# Autodesk Inventor assembly: HbHand
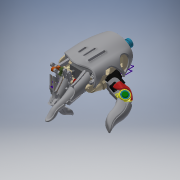
[picture p0: Inventor's stored thumbnail of the model, 180x180]
Saved by Autodesk Inventor 2017 (Build 210142000, 142)
## iProperties
Part Number: HbHand
Material: 一般
Document SubType Name: Assembly
Designer: sktom
Author: sktom
## Documents named in this file (20)
- D:\OneDrive\CAD\hackberry\HACKberry-hardware\3D_69%\HbHand\HbHand.iam
- D:\OneDrive\CAD\hackberry\HACKberry-hardware\3D_69%\HbHand\HbPalmBase03ForChild.ipt
- D:\OneDrive\CAD\hackberry\HACKberry-hardware\3D_69%\HbHand\HbWristMount01ForChild.ipt
- D:\OneDrive\CAD\hackberry\HACKberry-hardware\3D_69%\HbHand\DummyUsmBearing01.ipt
- D:\OneDrive\CAD\hackberry\HACKberry-hardware\3D_69%\HbHand\DummyASV-15MGSingleHorn01.ipt
- D:\OneDrive\CAD\hackberry\HACKberry-hardware\3D_69%\HbHand\HbthumbU02ForChild\HbthumbU02ForChild.iam
- D:\OneDrive\CAD\hackberry\HACKberry-hardware\3D_69%\HbHand\HbFinger01ForChild\HbFinger01ForChild.iam
- D:\OneDrive\CAD\hackberry\HACKberry-hardware\3D_69%\HbHand\HbShaftStopperB04ForChild.ipt
- D:\OneDrive\CAD\hackberry\HACKberry-hardware\3D_69%\HbHand\HbFingerMainCouplerLink01ForChild.ipt
- D:\OneDrive\CAD\hackberry\HACKberry-hardware\3D_69%\HbHand\DummyMetalCollarPh3L5.ipt
- D:\OneDrive\CAD\hackberry\HACKberry-hardware\3D_69%\HbHand\HbMiddle-RingCouplerLink01ForChild.ipt
- D:\OneDrive\CAD\hackberry\HACKberry-hardware\3D_69%\HbHand\HbRing-LittleCouplerLink01ForChild.ipt
- D:\OneDrive\CAD\hackberry\HACKberry-hardware\3D_69%\HbHand\HbIndexFinger01ForChild\HbIndexFinger01ForChild.iam
- D:\OneDrive\CAD\hackberry\HACKberry-hardware\3D_69%\HbHand\HbShaftStopperA04ForChild.ipt
- D:\OneDrive\CAD\hackberry\HACKberry-hardware\3D_69%\HbHand\DummyGWS_S03N.ipt
- D:\OneDrive\CAD\hackberry\HACKberry-hardware\3D_69%\HbHand\DummyHbServoHorn01.ipt
- D:\OneDrive\CAD\hackberry\HACKberry-hardware\3D_69%\HbHand\HbIndexMotorGear02ForChild.ipt
- D:\OneDrive\CAD\hackberry\HACKberry-hardware\3D_69%\HbHand\HbMotorHolder01ForChild.ipt
- D:\OneDrive\CAD\hackberry\HACKberry-hardware\3D_69%\HbHand\DummyASV-15MG.ipt
- D:\OneDrive\CAD\hackberry\HACKberry-hardware\3D_69%\HbHand\HbBackCover02ForChild.ipt
## Components (27 placed, 19 different names)
1. HbPalmBase03ForChild:1 — 挿入:1, 挿入:2, 挿入:3, 挿入:4, 挿入:5, 挿入:7, 円柱状:1, 挿入:8, 円柱状:2, 挿入:9, 円柱状:3, 挿入:10, 挿入:21, 挿入:22, 挿入:26, 挿入:27, 挿入:30, 挿入:31, 挿入:33, 挿入:34
2. HbWristMount01ForChild:1 — 挿入:1, 挿入:2
3. DummyUsmBearing01:1 — 挿入:3
4. DummyASV-15MGSingleHorn01:1 — 挿入:4, 挿入:5, 挿入:6
5. HbthumbU02ForChild:1 [sub-assembly] — 挿入:6
6. HbFinger01ForChild:1 [sub-assembly] — 挿入:7, 円柱状:1, 挿入:13, 円柱状:5
7. HbFinger01ForChild:2 [sub-assembly] — 挿入:8, 円柱状:2, 挿入:18, 挿入:20
8. HbFinger01ForChild:3 [sub-assembly] — 挿入:9, 円柱状:3, 円柱状:4
9. HbShaftStopperB04ForChild:1 — 挿入:10
10. HbFingerMainCouplerLink01ForChild:1 — 挿入:11, 挿入:12
11. DummyMetalCollarPh3L5:1 — 挿入:11, 挿入:13
12. DummyMetalCollarPh3L5:2 — 挿入:12, 円柱状:6
13. DummyMetalCollarPh3L5:3 — 挿入:16, 円柱状:5
14. DummyMetalCollarPh3L5:4 — 挿入:17, 挿入:18
15. DummyMetalCollarPh3L5:5 — 挿入:19, 挿入:20
16. DummyMetalCollarPh3L5:6 — 挿入:15, 円柱状:4
17. HbMiddle-RingCouplerLink01ForChild:1 — 挿入:15, 挿入:19
18. HbRing-LittleCouplerLink01ForChild:1 — 挿入:16, 挿入:17
19. HbIndexFinger01ForChild:1 [sub-assembly] — 挿入:21
20. HbShaftStopperA04ForChild:1 — 挿入:22
21. DummyGWS_S03N:1 — 挿入:25, 挿入:26, 挿入:27
22. DummyHbServoHorn01:1 — 挿入:23, 挿入:24, 挿入:25
23. HbIndexMotorGear02ForChild:1 — 挿入:23, 挿入:24
24. HbMotorHolder01ForChild:1 — 挿入:28, 挿入:29, 挿入:30, 挿入:31
25. DummyASV-15MG:1 — 挿入:28, 挿入:29, 挿入:32
26. DummyASV-15MGSingleHorn01:2 — 挿入:32, 円柱状:6
27. HbBackCover02ForChild:1 — 挿入:33, 挿入:34
## Relationships (39: Insert 33, CylindricalJoint 6)
- 挿入:1 [Insert]: HbPalmBase03ForChild:1 ↔ HbWristMount01ForChild:1
- 挿入:2 [Insert]: HbPalmBase03ForChild:1 ↔ HbWristMount01ForChild:1
- 挿入:3 [Insert]: HbPalmBase03ForChild:1 ↔ DummyUsmBearing01:1
- 挿入:4 [Insert]: HbPalmBase03ForChild:1 ↔ DummyASV-15MGSingleHorn01:1
- 挿入:5 [Insert]: HbPalmBase03ForChild:1 ↔ DummyASV-15MGSingleHorn01:1
- 挿入:6 [Insert]: DummyASV-15MGSingleHorn01:1 ↔ HbthumbU02ForChild:1
- 挿入:7 [Insert] (0.5 mm): HbPalmBase03ForChild:1 ↔ HbFinger01ForChild:1
- 円柱状:1 [CylindricalJoint]: HbPalmBase03ForChild:1 ↔ HbFinger01ForChild:1
- 挿入:8 [Insert] (0.5 mm): HbPalmBase03ForChild:1 ↔ HbFinger01ForChild:2
- 円柱状:2 [CylindricalJoint]: HbPalmBase03ForChild:1 ↔ HbFinger01ForChild:2
- 挿入:9 [Insert] (0.5 mm): HbPalmBase03ForChild:1 ↔ HbFinger01ForChild:3
- 円柱状:3 [CylindricalJoint]: HbPalmBase03ForChild:1 ↔ HbFinger01ForChild:3
- 挿入:10 [Insert]: HbPalmBase03ForChild:1 ↔ HbShaftStopperB04ForChild:1
- 挿入:11 [Insert] (-0.5 mm): HbFingerMainCouplerLink01ForChild:1 ↔ DummyMetalCollarPh3L5:1
- 挿入:12 [Insert] (-0.5 mm): HbFingerMainCouplerLink01ForChild:1 ↔ DummyMetalCollarPh3L5:2
- 挿入:13 [Insert]: HbFinger01ForChild:1 ↔ DummyMetalCollarPh3L5:1
- 挿入:15 [Insert] (-0.2 mm): DummyMetalCollarPh3L5:6 ↔ HbMiddle-RingCouplerLink01ForChild:1
- 挿入:16 [Insert]: DummyMetalCollarPh3L5:3 ↔ HbRing-LittleCouplerLink01ForChild:1
- 挿入:17 [Insert]: DummyMetalCollarPh3L5:4 ↔ HbRing-LittleCouplerLink01ForChild:1
- 挿入:18 [Insert]: HbFinger01ForChild:2 ↔ DummyMetalCollarPh3L5:4
- 挿入:19 [Insert]: DummyMetalCollarPh3L5:5 ↔ HbMiddle-RingCouplerLink01ForChild:1
- 挿入:20 [Insert]: HbFinger01ForChild:2 ↔ DummyMetalCollarPh3L5:5
- 円柱状:4 [CylindricalJoint]: HbFinger01ForChild:3 ↔ DummyMetalCollarPh3L5:6
- 円柱状:5 [CylindricalJoint]: HbFinger01ForChild:1 ↔ DummyMetalCollarPh3L5:3
- 挿入:21 [Insert] (0.25 mm): HbPalmBase03ForChild:1 ↔ HbIndexFinger01ForChild:1
- 挿入:22 [Insert]: HbPalmBase03ForChild:1 ↔ HbShaftStopperA04ForChild:1
- 挿入:23 [Insert]: DummyHbServoHorn01:1 ↔ HbIndexMotorGear02ForChild:1
- 挿入:24 [Insert]: DummyHbServoHorn01:1 ↔ HbIndexMotorGear02ForChild:1
- 挿入:25 [Insert]: DummyGWS_S03N:1 ↔ DummyHbServoHorn01:1
- 挿入:26 [Insert]: HbPalmBase03ForChild:1 ↔ DummyGWS_S03N:1
- 挿入:27 [Insert]: HbPalmBase03ForChild:1 ↔ DummyGWS_S03N:1
- 挿入:28 [Insert]: HbMotorHolder01ForChild:1 ↔ DummyASV-15MG:1
- 挿入:29 [Insert]: HbMotorHolder01ForChild:1 ↔ DummyASV-15MG:1
- 挿入:30 [Insert]: HbPalmBase03ForChild:1 ↔ HbMotorHolder01ForChild:1
- 挿入:31 [Insert]: HbPalmBase03ForChild:1 ↔ HbMotorHolder01ForChild:1
- 挿入:32 [Insert]: DummyASV-15MG:1 ↔ DummyASV-15MGSingleHorn01:2
- 円柱状:6 [CylindricalJoint]: DummyMetalCollarPh3L5:2 ↔ DummyASV-15MGSingleHorn01:2
- 挿入:33 [Insert]: HbPalmBase03ForChild:1 ↔ HbBackCover02ForChild:1
- 挿入:34 [Insert]: HbPalmBase03ForChild:1 ↔ HbBackCover02ForChild:1
